# Autodesk Inventor assembly: chamber_assembly_V2
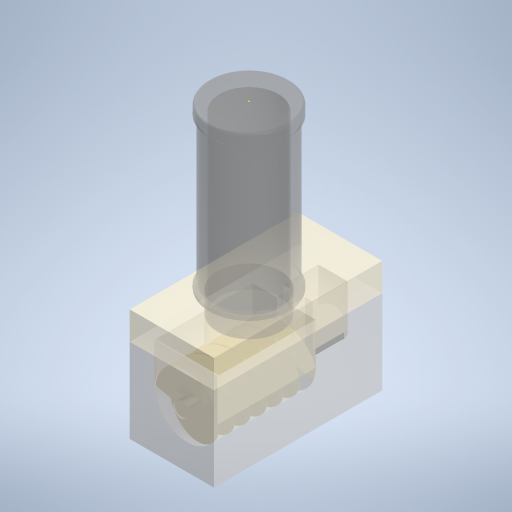
[picture p0: Inventor's stored thumbnail of the model, 512x512]
Saved by Autodesk Inventor 2023 (Build 270158000, 158)
## iProperties
Created: 2023-03-23
Part Number: chamber_assembly_V2
Document SubType Name: Assembly
Designer: caleb
Author: caleb
## Documents named in this file (6)
- C:\Users\caleb\Documents\Inventor\SPICE\chamber_assembly_V2.iam
- C:\Users\caleb\Documents\Inventor\SPICE\housing_V2.ipt
- C:\Users\caleb\Documents\Inventor\SPICE\housing_lid_V2.ipt
- C:\Users\caleb\Documents\Inventor\SPICE\FiestaSpiceContainer.ipt
- C:\Users\caleb\Documents\Inventor\SPICE\DCMotorAssembly.iam
- C:\Users\caleb\Documents\Inventor\SPICE\spiral.ipt
## Components (5 placed, 5 different names)
1. housing_V2:1 — Flush:1, Flush:2, Mate:3, Mate:4, Mate:5, Mate:6, Mate:7
2. housing_lid_V2:1 — Flush:1, Flush:2, Mate:1, Mate:2, Mate:7
3. FiestaSpiceContainer:1 — Mate:1, Mate:2
4. DCMotorAssembly:1 [sub-assembly] — Mate:3, Mate:4
5. spiral:1 — Mate:5, Mate:6
## Relationships (9: Mate 7, Flush 2)
- Flush:1: housing_V2:1 ↔ housing_lid_V2:1
- Flush:2: housing_V2:1 ↔ housing_lid_V2:1
- Mate:1: housing_lid_V2:1 ↔ FiestaSpiceContainer:1
- Mate:2: housing_lid_V2:1 ↔ FiestaSpiceContainer:1
- Mate:3: housing_V2:1 ↔ DCMotorAssembly:1
- Mate:4: housing_V2:1 ↔ DCMotorAssembly:1
- Mate:5: housing_V2:1 ↔ spiral:1
- Mate:6: housing_V2:1 ↔ spiral:1
- Mate:7: housing_V2:1 ↔ housing_lid_V2:1
